# Autodesk Inventor assembly: Leg
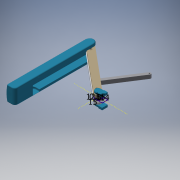
[picture p0: Inventor's stored thumbnail of the model, 180x180]
Saved by Autodesk Inventor 2019.1 (Build 231200000, 200)
## iProperties
Created: 2018-10-31
Part Number: Leg
Material: Generisch
Document SubType Name: Assembly
Designer: JochenAlt
Author: JochenAlt
## Documents named in this file (7)
- D:\Projects\Ondine\CAD\Leg\Leg.iam
- D:\Projects\Ondine\CAD\Leg\Hip.ipt
- D:\Projects\Ondine\CAD\Leg\Knee.ipt
- D:\Projects\Ondine\CAD\Leg\Thigh.ipt
- D:\Projects\Ondine\CAD\Leg\LegConstruction\Konstruktions-Assistent\Zahnriemen1.ipt
- C:\Users\JochenAlt\Documents\Inventor\Content Center Files\R2019\de-DE\BS 290 SKF(30)\BS 290 SKF - SKF 618_5.ipt
- D:\Projects\Ondine\CAD\Leg\Lever.ipt
## Components (9 placed, 5 different names)
1. Hip:1 — Passend:4, Passend:5, Passend:10, Passend:11, Passend:19, Winkel:4, Passend:28
2. Hip:2 — Passend:6, Passend:7, Passend:8, Passend:13, Passend:14, Winkel:4
3. Thigh:1 — Passend:12, Passend:15, Passend:16, Passend:19, Passend:24, Passend:25, Passend:26, Passend:27, Winkel:7
4. Zahnriemen:1 — Passend:26, Passend:27, Winkel:7
5. BS 290 SKF 618/5:1 — Passend:4, Passend:5
6. BS 290 SKF 618/5:2 — Passend:6, Passend:7, Passend:16
7. BS 290 SKF 618/5:3 — Passend:8, Passend:13, Passend:14, Passend:15
8. BS 290 SKF 618/5:4 — Passend:10, Passend:11, Passend:12
9. Lever:1 — Passend:24, Passend:25, Passend:28
## Relationships (20: Mate 18, Angle 2)
- Passend:4 [Mate]: Hip:1 ↔ BS 290 SKF 618/5:1
- Passend:5 [Mate]: Hip:1 ↔ BS 290 SKF 618/5:1
- Passend:6 [Mate]: Hip:2 ↔ BS 290 SKF 618/5:2
- Passend:7 [Mate]: Hip:2 ↔ BS 290 SKF 618/5:2
- Passend:8 [Mate]: Hip:2 ↔ BS 290 SKF 618/5:3
- Passend:10 [Mate]: Hip:1 ↔ BS 290 SKF 618/5:4
- Passend:11 [Mate]: Hip:1 ↔ BS 290 SKF 618/5:4
- Passend:12 [Mate]: Thigh:1 ↔ BS 290 SKF 618/5:4
- Passend:13 [Mate]: Hip:2 ↔ BS 290 SKF 618/5:3
- Passend:14 [Mate]: Hip:2 ↔ BS 290 SKF 618/5:3
- Passend:15 [Mate]: Thigh:1 ↔ BS 290 SKF 618/5:3
- Passend:16 [Mate]: Thigh:1 ↔ BS 290 SKF 618/5:2
- Passend:19 [Mate]: Hip:1 ↔ Thigh:1
- Winkel:4 [Angle] (0 deg): Hip:1 ↔ Hip:2
- Passend:24 [Mate]: Thigh:1 ↔ Lever:1
- Passend:25 [Mate] (0.5 mm): Thigh:1 ↔ Lever:1
- Passend:26 [Mate]: Thigh:1 ↔ Zahnriemen:1
- Passend:27 [Mate] (1.5 mm): Thigh:1 ↔ Zahnriemen:1
- Winkel:7 [Angle] (0 deg): Thigh:1 ↔ Zahnriemen:1
- Passend:28 [Mate]: Hip:1 ↔ Lever:1
